# Autodesk Inventor assembly: CO-0-1-BatteryUnit
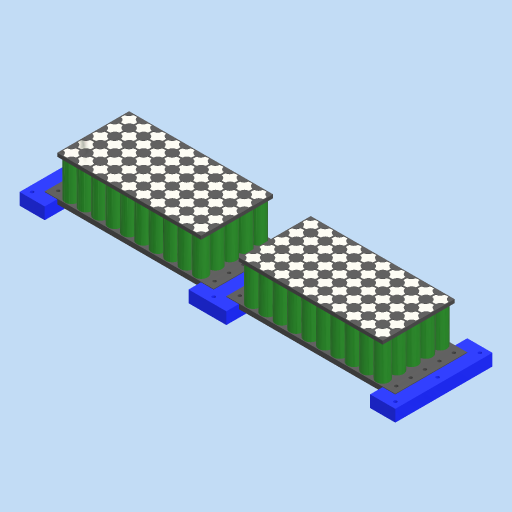
[picture p0: Inventor's stored thumbnail of the model, 512x512]
Saved by Autodesk Inventor 2023 (Build 270158000, 158)
## iProperties
Created: 2023-01-22
Part Number: CO-0-1-BatteryUnit
Document SubType Name: Assembly
Designer: asach
Author: asach
## Documents named in this file (6)
- C:\Github\BehrendURC\CAD\Controls\CO-0-1-BatteryUnit.iam
- C:\Github\BehrendURC\CAD\Controls\CO-2-1_CellSpacerBottom.ipt
- C:\Github\BehrendURC\CAD\Controls\CO-1-1-BatteryCell.ipt
- C:\Github\BehrendURC\CAD\Controls\CO-1-1_CellSpacer10by5.ipt
- C:\Github\BehrendURC\CAD\Controls\CO-1-1-CellSpacerMount.ipt
- C:\Github\BehrendURC\CAD\Controls\CO-1-1-CellSpacerMountMiddle.ipt
## Components (107 placed, 5 different names)
1. CO-2-1_CellSpacerBottom:1 — Mate:1, Mate:2, Mate:6, Mate:7, Mate:8, Mate:9, Mate:10
2. CO-1-1_CellSpacer10by5:1 — Mate:3, Mate:4, Mate:5
3. CO-1-1-CellSpacerMount:1 — Mate:6, Mate:7, Mate:8
4. CO-1-1-CellSpacerMountMiddle:1 — Mate:9, Mate:10, Mate:11, Mate:12, Mate:13
5. CO-2-1_CellSpacerBottom:2 — Mate:11, Mate:12, Mate:13, Mate:14, Mate:15, Mate:18, Mate:19, Mate:20
6. CO-1-1_CellSpacer10by5:2 — Mate:16, Mate:17
7. CO-1-1-CellSpacerMount:2 — Mate:18, Mate:19, Mate:20
8. CO-1-1-BatteryCell:1 — Mate:1, Mate:2, Mate:5
9. CO-1-1-BatteryCell:2
10. CO-1-1-BatteryCell:3
11. CO-1-1-BatteryCell:4
12. CO-1-1-BatteryCell:5
13. CO-1-1-BatteryCell:6
14. CO-1-1-BatteryCell:7
15. CO-1-1-BatteryCell:8
16. CO-1-1-BatteryCell:9
17. CO-1-1-BatteryCell:10
18. CO-1-1-BatteryCell:11
19. CO-1-1-BatteryCell:12
20. CO-1-1-BatteryCell:13
21. CO-1-1-BatteryCell:14
22. CO-1-1-BatteryCell:15
23. CO-1-1-BatteryCell:16
24. CO-1-1-BatteryCell:17
25. CO-1-1-BatteryCell:18
26. CO-1-1-BatteryCell:19
27. CO-1-1-BatteryCell:20
28. CO-1-1-BatteryCell:21
29. CO-1-1-BatteryCell:22
30. CO-1-1-BatteryCell:23
31. CO-1-1-BatteryCell:24
32. CO-1-1-BatteryCell:25
33. CO-1-1-BatteryCell:26
34. CO-1-1-BatteryCell:27
35. CO-1-1-BatteryCell:28
36. CO-1-1-BatteryCell:29
37. CO-1-1-BatteryCell:30
38. CO-1-1-BatteryCell:31
39. CO-1-1-BatteryCell:32
40. CO-1-1-BatteryCell:33
41. CO-1-1-BatteryCell:34
42. CO-1-1-BatteryCell:35
43. CO-1-1-BatteryCell:36
44. CO-1-1-BatteryCell:37
45. CO-1-1-BatteryCell:38
46. CO-1-1-BatteryCell:39
47. CO-1-1-BatteryCell:40
48. CO-1-1-BatteryCell:41
49. CO-1-1-BatteryCell:42
50. CO-1-1-BatteryCell:43
51. CO-1-1-BatteryCell:44
52. CO-1-1-BatteryCell:45
53. CO-1-1-BatteryCell:46
54. CO-1-1-BatteryCell:47
55. CO-1-1-BatteryCell:48
56. CO-1-1-BatteryCell:49
57. CO-1-1-BatteryCell:50 — Mate:3, Mate:4
58. CO-1-1-BatteryCell:51 — Mate:14, Mate:15, Mate:16, Mate:17
59. CO-1-1-BatteryCell:52
60. CO-1-1-BatteryCell:53
61. CO-1-1-BatteryCell:54
62. CO-1-1-BatteryCell:55
63. CO-1-1-BatteryCell:56
64. CO-1-1-BatteryCell:57
65. CO-1-1-BatteryCell:58
66. CO-1-1-BatteryCell:59
67. CO-1-1-BatteryCell:60
68. CO-1-1-BatteryCell:61
69. CO-1-1-BatteryCell:62
70. CO-1-1-BatteryCell:63
71. CO-1-1-BatteryCell:64
72. CO-1-1-BatteryCell:65
73. CO-1-1-BatteryCell:66
74. CO-1-1-BatteryCell:67
75. CO-1-1-BatteryCell:68
76. CO-1-1-BatteryCell:69
77. CO-1-1-BatteryCell:70
78. CO-1-1-BatteryCell:71
79. CO-1-1-BatteryCell:72
80. CO-1-1-BatteryCell:73
81. CO-1-1-BatteryCell:74
82. CO-1-1-BatteryCell:75
83. CO-1-1-BatteryCell:76
84. CO-1-1-BatteryCell:77
85. CO-1-1-BatteryCell:78
86. CO-1-1-BatteryCell:79
87. CO-1-1-BatteryCell:80
88. CO-1-1-BatteryCell:81
89. CO-1-1-BatteryCell:82
90. CO-1-1-BatteryCell:83
91. CO-1-1-BatteryCell:84
92. CO-1-1-BatteryCell:85
93. CO-1-1-BatteryCell:86
94. CO-1-1-BatteryCell:87
95. CO-1-1-BatteryCell:88
96. CO-1-1-BatteryCell:89
97. CO-1-1-BatteryCell:90
98. CO-1-1-BatteryCell:91
99. CO-1-1-BatteryCell:92
100. CO-1-1-BatteryCell:93
101. CO-1-1-BatteryCell:94
102. CO-1-1-BatteryCell:95
103. CO-1-1-BatteryCell:96
104. CO-1-1-BatteryCell:97
105. CO-1-1-BatteryCell:98
106. CO-1-1-BatteryCell:99
107. CO-1-1-BatteryCell:100
## Component patterns: (50 elements, first: CO-1-1-BatteryCell:1), (50 elements, first: CO-1-1-BatteryCell:51)
## Relationships (20: Mate 20)
- Mate:1: CO-2-1_CellSpacerBottom:1 ↔ CO-1-1-BatteryCell:1
- Mate:2: CO-2-1_CellSpacerBottom:1 ↔ CO-1-1-BatteryCell:1
- Mate:3: CO-1-1_CellSpacer10by5:1 ↔ CO-1-1-BatteryCell:50
- Mate:4: CO-1-1_CellSpacer10by5:1 ↔ CO-1-1-BatteryCell:50
- Mate:5: CO-1-1_CellSpacer10by5:1 ↔ CO-1-1-BatteryCell:1
- Mate:6: CO-2-1_CellSpacerBottom:1 ↔ CO-1-1-CellSpacerMount:1
- Mate:7: CO-2-1_CellSpacerBottom:1 ↔ CO-1-1-CellSpacerMount:1
- Mate:8: CO-2-1_CellSpacerBottom:1 ↔ CO-1-1-CellSpacerMount:1
- Mate:9: CO-2-1_CellSpacerBottom:1 ↔ CO-1-1-CellSpacerMountMiddle:1
- Mate:10: CO-2-1_CellSpacerBottom:1 ↔ CO-1-1-CellSpacerMountMiddle:1
- Mate:11: CO-1-1-CellSpacerMountMiddle:1 ↔ CO-2-1_CellSpacerBottom:2
- Mate:12: CO-1-1-CellSpacerMountMiddle:1 ↔ CO-2-1_CellSpacerBottom:2
- Mate:13: CO-1-1-CellSpacerMountMiddle:1 ↔ CO-2-1_CellSpacerBottom:2
- Mate:14: CO-2-1_CellSpacerBottom:2 ↔ CO-1-1-BatteryCell:51
- Mate:15: CO-2-1_CellSpacerBottom:2 ↔ CO-1-1-BatteryCell:51
- Mate:16: CO-1-1_CellSpacer10by5:2 ↔ CO-1-1-BatteryCell:51
- Mate:17: CO-1-1_CellSpacer10by5:2 ↔ CO-1-1-BatteryCell:51
- Mate:18: CO-2-1_CellSpacerBottom:2 ↔ CO-1-1-CellSpacerMount:2
- Mate:19: CO-2-1_CellSpacerBottom:2 ↔ CO-1-1-CellSpacerMount:2
- Mate:20: CO-2-1_CellSpacerBottom:2 ↔ CO-1-1-CellSpacerMount:2
